# Autodesk Inventor assembly: 6P Sprocket
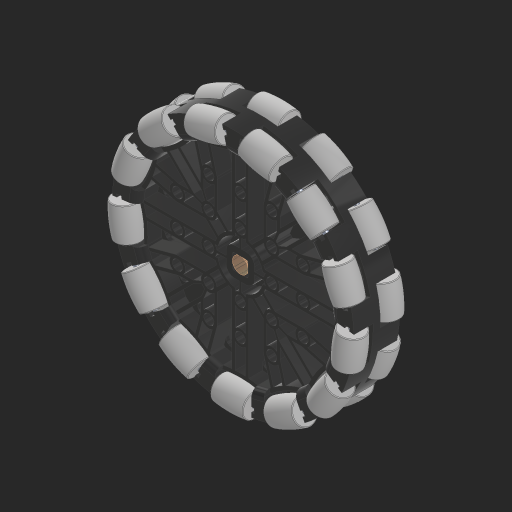
[picture p0: Inventor's stored thumbnail of the model, 512x512]
Saved by Autodesk Inventor 2023 (Build 270158000, 158)
## iProperties
Created: 2022-08-02
Part Number: 6P Sprocket
Document SubType Name: Assembly
Designer: ylu12
Author: ylu12
## Documents named in this file (3)
- C:\Users\ylu12\Documents\GitHub\VEX-CAD-Inventor\Motion\Wheels\Omni Wheel\4 Omni AS, No Insert.iam
- C:\Users\ylu12\Documents\GitHub\VEX-CAD-Inventor\Motion\Wheels\Reference Files\4 Omni Antistatic.ipt
- C:\Users\ylu12\Documents\GitHub\VEX-CAD-Inventor\Motion\Wheels\Omni Wheel.iam
## Components (1 placed, 1 different names)
1. 4 Omni Antistatic
## Relationships (3: Mate 2, Flush 1)
- [Flush]: 4 Omni Antistatic
- [Mate]: 4 Omni Antistatic
- [Mate]: 4 Omni Antistatic
